# Autodesk Inventor assembly: teljes3
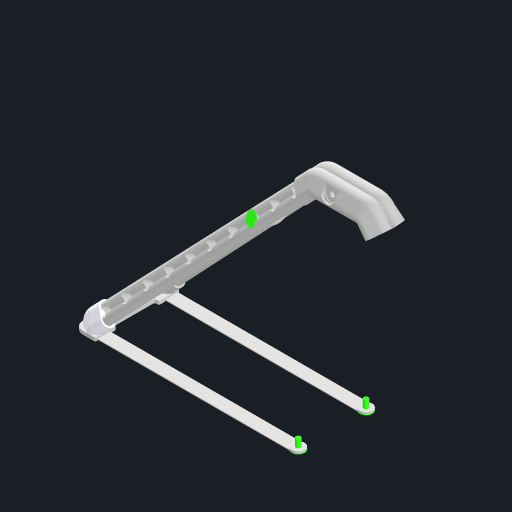
[picture p0: Inventor's stored thumbnail of the model, 512x512]
Saved by Autodesk Inventor 2023 (Build 270158000, 158)
## iProperties
Created: 2022-11-11
Part Number: teljes3
Document SubType Name: Assembly
Designer: gd1
Author: gd1
## Documents named in this file (8)
- C:\Users\gd1\3D Objects\3D nagyteherbírású híd\Híd\H-d\teljes7.iam
- C:\Users\gd1\3D Objects\3D nagyteherbírású híd\Híd\H-d\palca 325mm.ipt
- C:\Users\gd1\3D Objects\3D nagyteherbírású híd\Híd\H-d\tipli.ipt
- C:\Users\gd1\3D Objects\3D nagyteherbírású híd\Híd\H-d\45 fok középre_talp másolata.ipt
- C:\Users\gd1\3D Objects\3D nagyteherbírású híd\Híd\H-d\osszekotoelem.iam
- C:\Users\gd1\3D Objects\3D nagyteherbírású híd\Híd\H-d\45 fok kozepcsati.ipt.iam
- C:\Users\gd1\3D Objects\3D nagyteherbírású híd\Híd\H-d\kozepso szalag2.ipt
- 45 fok kozepcsati.ipt
## Components (13 placed, 6 different names)
1. palca 325mm:1 — Rotational:5, Rotational:6
2. palca 325mm:2 — Rotational:9
3. tipli:1
4. tipli:2
5. 45 fok középre_talp másolata:1 — Rotational:5, Rotational:10, Rotational:11
6. osszekotoelem:1 [sub-assembly] — Rotational:6, Rotational:7, Rotational:8
7. tipli:3 — Rotational:7
8. tipli:4 — Rotational:8
9. 45 fok kozepcsati.ipt:1 [sub-assembly] — Rotational:9
10. kozepso szalag2:1 — Rotational:10, Rigid:1
11. kozepso szalag2:2 — Rotational:11, Rigid:2
12. tipli:5 — Rigid:1
13. tipli:6 — Rigid:2
## Relationships (9: RevoluteJoint 7, WeldJoint 2)
- Rotational:5 [RevoluteJoint]: palca 325mm:1 ↔ 45 fok középre_talp másolata:1
- Rotational:6 [RevoluteJoint]: palca 325mm:1 ↔ osszekotoelem:1
- Rotational:7 [RevoluteJoint]: osszekotoelem:1 ↔ tipli:3
- Rotational:8 [RevoluteJoint]: osszekotoelem:1 ↔ tipli:4
- Rotational:9 [RevoluteJoint]: palca 325mm:2 ↔ 45 fok kozepcsati.ipt:1
- Rotational:10 [RevoluteJoint]: 45 fok középre_talp másolata:1 ↔ kozepso szalag2:1
- Rotational:11 [RevoluteJoint]: 45 fok középre_talp másolata:1 ↔ kozepso szalag2:2
- Rigid:1 [WeldJoint]: kozepso szalag2:1 ↔ tipli:5
- Rigid:2 [WeldJoint]: kozepso szalag2:2 ↔ tipli:6
